# Autodesk Inventor assembly: Assembly1
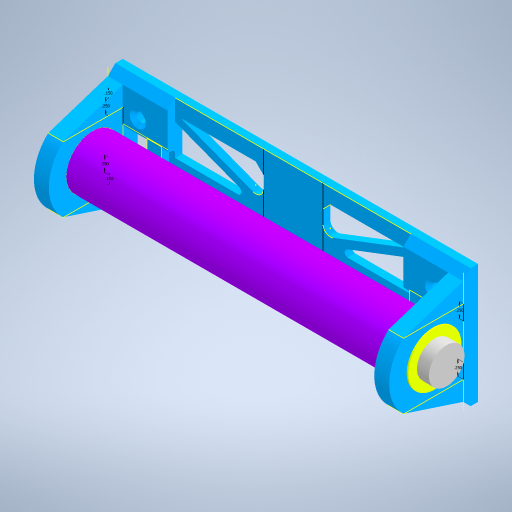
[picture p0: Inventor's stored thumbnail of the model, 512x512]
Saved by Autodesk Inventor 2023 (Build 270158030, 158C)
## iProperties
Created: 2022-10-15
Part Number: Assembly1
Document SubType Name: Assembly
Designer: rm0990889
Author: rm0990889
## Documents named in this file (5)
- C:\Users\rm0990889\Downloads\Belt-Tensioner-CAD-main\Belt-Tensioner-CAD-main\Assembly1.iam
- C:\Users\rm0990889\Downloads\Belt-Tensioner-CAD-main\Belt-Tensioner-CAD-main\belt tensioner base.ipt
- C:\Users\rm0990889\Downloads\Belt-Tensioner-CAD-main\Belt-Tensioner-CAD-main\small bearing.ipt
- C:\Users\rm0990889\Downloads\Belt-Tensioner-CAD-main\Belt-Tensioner-CAD-main\roller.ipt
- C:\Users\rm0990889\Downloads\Belt-Tensioner-CAD-main\Belt-Tensioner-CAD-main\roller pin.ipt
## Components (5 placed, 4 different names)
1. belt tensioner base:1 — Mate:1, Mate:2, Flush:2, Flush:3
2. small bearing:1 — Mate:2, Flush:2
3. small bearing:2 — Mate:1, Flush:3, Insert:1, Flush:4, Insert:2
4. roller:1 — Insert:1
5. roller pin:1 — Flush:4, Insert:2
## Relationships (7: Flush 3, Mate 2, Insert 2)
- Mate:1: belt tensioner base:1 ↔ small bearing:2
- Mate:2: belt tensioner base:1 ↔ small bearing:1
- Flush:2: belt tensioner base:1 ↔ small bearing:1
- Flush:3: belt tensioner base:1 ↔ small bearing:2
- Insert:1: small bearing:2 ↔ roller:1
- Flush:4: small bearing:2 ↔ roller pin:1
- Insert:2: small bearing:2 ↔ roller pin:1
